# Autodesk Inventor assembly: servo
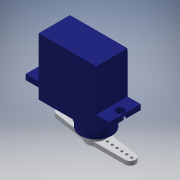
[picture p0: Inventor's stored thumbnail of the model, 180x180]
Saved by Autodesk Inventor 2016 (Build 200138000, 138)
## iProperties
Created: 2017-12-29
Part Number: servo
Material: Genérico
Document SubType Name: Assembly
Designer: David
Author: David
## Documents named in this file (3)
- C:\Users\David\Desktop\robot1 2018\piezas\servo.iam
- C:\Users\David\Desktop\robot1 2018\piezas\cosito servo.ipt
- C:\Users\David\Desktop\robot1 2018\piezas\servo.ipt
## Components (2 placed, 2 different names)
1. cosito servo:1 — De rotación:1
2. servo:1 — De rotación:1
## Relationships (1: RevoluteJoint 1)
- De rotación:1 [RevoluteJoint]: cosito servo:1 ↔ servo:1
